# Autodesk Inventor assembly: Assembly Plate Assembly
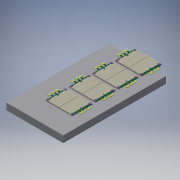
[picture p0: Inventor's stored thumbnail of the model, 180x180]
Saved by Autodesk Inventor 2019.4 (Build 234330000, 330)
## iProperties
Created: 2021-01-11
Part Number: Assembly Plate Assembly
Document SubType Name: Assembly
Designer: caleb
Author: caleb
## Documents named in this file (3)
- C:\Users\cfang\Desktop\nebraska-silicon-lab\CAD\ETL\Module Assembly\Assembly Plate\Assembly Plate Assembly.iam
- C:\Users\cfang\Desktop\nebraska-silicon-lab\CAD\ETL\Module Assembly\Assembly Plate\Assembly Plate.ipt
- C:\Users\cfang\Desktop\nebraska-silicon-lab\CAD\ETL\modules\tdr\F10110887--_1-MODULE_ CMS2 ETL_ FULL DBL-SENSOR MOUNTED ASSY.ipt
## Components (5 placed, 2 different names)
1. Assembly Plate:1 — Mate:1, Flush:1, Mate:2, Mate:3, Mate:4
2. F10110887--_1-MODULE_ CMS2 ETL_ FULL DBL-SENSOR MOUNTED ASSY:1 — Mate:1, Flush:1
3. F10110887--_1-MODULE_ CMS2 ETL_ FULL DBL-SENSOR MOUNTED ASSY:2 — Mate:2
4. F10110887--_1-MODULE_ CMS2 ETL_ FULL DBL-SENSOR MOUNTED ASSY:3 — Mate:4
5. F10110887--_1-MODULE_ CMS2 ETL_ FULL DBL-SENSOR MOUNTED ASSY:4 — Mate:3
## Relationships (5: Mate 4, Flush 1)
- Mate:1: Assembly Plate:1 ↔ F10110887--_1-MODULE_ CMS2 ETL_ FULL DBL-SENSOR MOUNTED ASSY:1
- Flush:1 (25.4 mm): Assembly Plate:1 ↔ F10110887--_1-MODULE_ CMS2 ETL_ FULL DBL-SENSOR MOUNTED ASSY:1
- Mate:2: Assembly Plate:1 ↔ F10110887--_1-MODULE_ CMS2 ETL_ FULL DBL-SENSOR MOUNTED ASSY:2
- Mate:3: Assembly Plate:1 ↔ F10110887--_1-MODULE_ CMS2 ETL_ FULL DBL-SENSOR MOUNTED ASSY:4
- Mate:4: Assembly Plate:1 ↔ F10110887--_1-MODULE_ CMS2 ETL_ FULL DBL-SENSOR MOUNTED ASSY:3
